# Autodesk Inventor assembly: wafel_rev2
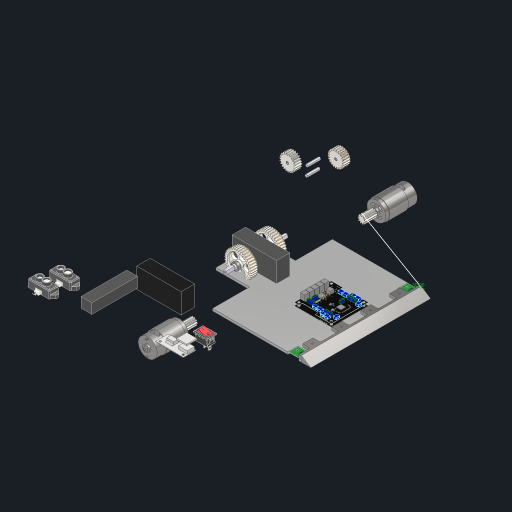
[picture p0: Inventor's stored thumbnail of the model, 512x512]
Saved by Autodesk Inventor 2023 (Build 270158000, 158)
## iProperties
Created: 2024-04-29
Part Number: wafel_rev2
Document SubType Name: Assembly
Designer: szymo
Mass: 970.153 g
Surface Area: 2764.06 cm^2
Volume: 500.252 cm^3
Density: 1.93933 g/cm^3
Author: szymo
## iProperties of the stored document TFMINI_S_UART.ipt
Created: 2023-12-04
Part Number: TFMINI S UART
Material: Generic
Description: STEP AP214
Document SubType Name: Modeling
Designer: mateu
Density: 1 g/cm^3
Appearance: Default
Sending System: SolidWorks 2016
Preprocessor: SwSTEP 2.0
Title: TFMINI S UART.STEP
Author: USER
Revision Number: ANY
## Documents named in this file (17)
- D:\roboilo\robots\codename wafel - australia\3d_parts\rev3\wafel_rev3.iam
- D:\roboilo\robots\codename wafel - australia\3d_parts\rev3\plog.ipt
- D:\roboilo\robots\codename wafel - australia\3d_parts\rev3\smolgear_shaft.ipt
- D:\roboilo\robots\codename wafel - australia\3d_parts\rev3\smolLipo.ipt
- D:\roboilo\robots\codename wafel - australia\3d_parts\rev3\stack.iam
- D:\roboilo\robots\codename wafel - australia\3d_parts\rev3\Switch.ipt
- D:\roboilo\robots\codename wafel - australia\3d_parts\rev3\wheel_axle.iam
- D:\roboilo\robots\codename wafel - australia\3d_parts\rev3\KTIR-Board.ipt
- D:\roboilo\robots\codename wafel - australia\3d_parts\rev3\lipo3s650.ipt
- D:\roboilo\robots\codename wafel - australia\3d_parts\rev3\Design Accelerator\smolGear.iam
- D:\roboilo\robots\codename wafel - australia\3d_parts\rev3\motor_w_gear.iam
- D:\roboilo\robots\codename wafel - australia\3d_parts\rev3\base.ipt
- D:\roboilo\robots\codename wafel - australia\3d_parts\rev3\wheel.ipt
- D:\roboilo\robots\codename wafel - australia\3d_parts\rev3\interface_board.ipt
- D:\roboilo\robots\codename wafel - australia\3d_parts\rev3\oled.ipt
- **D:\roboilo\robots\codename wafel - australia\3d_parts\rev3\wafel_rev3.iam*LocalDocs*xAaaaqfaaAaaaaaaaAaaaqmipFc*TFMINI_S_UART.ipt
- D:\roboilo\robots\codename wafel - australia\3d_parts\rev3\TFMINI_S_UART.ipt
## Components (23 placed, 16 different names)
1. base:1 — Mate:1, Flush:1, Mate:3, Mate:4, Flush:2, Mate:5, Mate:6, Flush:3, Mate:7, Flush:4, Flush:5, Mate:8, Angle:1, Mate:9
2. plog:1 — Mate:2
3. wheel_axle:1 [sub-assembly] — Mate:8, Angle:1, Mate:11
4. smolGear:1 [sub-assembly]
5. wheel:1
6. motor_w_gear:1 [sub-assembly]
7. motor_w_gear:2 [sub-assembly]
8. wheel_axle:2 [sub-assembly] — Mate:9, Mate:10
9. smolGear:2 [sub-assembly]
10. wheel:2
11. smolLipo:1
12. smolgear_shaft:1
13. smolgear_shaft:2
14. stack:1 [sub-assembly] — Mate:1, Flush:1, Mate:2
15. Switch:1
16. KTIR-Board:1 — Mate:3, Mate:4, Flush:2
17. KTIR-Board:2 — Mate:5, Mate:6, Flush:3
18. interface_board:1
19. oled:1
20. BIGlipo3s650:1 — Mate:7, Flush:4, Flush:5, Mate:10, Mate:11
21. lipo3s650:2
22. TFMINI_S_UART:1
23. TFMINI_S_UART:2
## Relationships (17: Mate 11, Flush 5, Angle 1)
- Mate:1 (2 mm): base:1 ↔ stack:1
- Flush:1 (61.5 mm): base:1 ↔ stack:1
- Mate:2 (2 mm): plog:1 ↔ stack:1
- Mate:3 (0.5 mm): base:1 ↔ KTIR-Board:1
- Mate:4 (0.5 mm): base:1 ↔ KTIR-Board:1
- Flush:2: base:1 ↔ KTIR-Board:1
- Mate:5 (0.5 mm): base:1 ↔ KTIR-Board:2
- Mate:6 (0.5 mm): base:1 ↔ KTIR-Board:2
- Flush:3: base:1 ↔ KTIR-Board:2
- Mate:7: base:1 ↔ BIGlipo3s650:1
- Flush:4: base:1 ↔ BIGlipo3s650:1
- Flush:5 (79 mm): base:1 ↔ BIGlipo3s650:1
- Mate:8 (-25 mm): base:1 ↔ wheel_axle:1
- Angle:1 (0 deg): base:1 ↔ wheel_axle:1
- Mate:9 (-25 mm): base:1 ↔ wheel_axle:2
- Mate:10 (1 mm): wheel_axle:2 ↔ BIGlipo3s650:1
- Mate:11 (1 mm): wheel_axle:1 ↔ BIGlipo3s650:1
